# Autodesk Inventor assembly: 000 Ensamblaje hw_DAA - PCB Peripherals
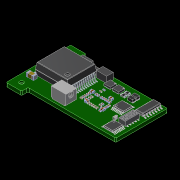
[picture p0: Inventor's stored thumbnail of the model, 180x180]
Saved by Autodesk Inventor 2018 (Build 220112000, 112)
## iProperties
Created: 2024-03-13
Part Number: 000 Ensamblaje hw_DAA - PCB Peripherals
Document SubType Name: Assembly
Designer: cda1
Author: cda1
## Documents named in this file (38)
- C:\Users\cda1\Git\DAA\items\hw_DAA\variants\BASIC\3d\000 Ensamblaje hw_DAA - PCB Peripherals.iam
- C:\Users\cda1\Git\DAA\items\hw_DAA\3d\hw_DAA - PCB Peripherals.ipt
- C:\Users\cda1\Git\DAA\items\_accessories\Componentes PCB\Drivers\3d_Texas Instruments\3d\SN65C3221IPWRQ1\SN65C3221IPWRQ1.iam
- C:\Users\cda1\Git\DAA\items\_accessories\Componentes PCB\Drivers\3d_Texas Instruments\3d\SN65HVD33MDREP\SN65HVD33MDREP.iam
- C:\Users\cda1\Git\DAA\items\_accessories\Componentes PCB\CAN\3d\3d_Texas_Instruments\TCAN1462VDRBRQ1\TCAN1462VDRBRQ1.iam
- C:\Users\cda1\Git\DAA\items\_accessories\Componentes PCB\Optoacoplador\3d_Toshiba\3d\TLP3431\TLP3431_TP,F.iam
- C:\Users\cda1\Git\DAA\items\_accessories\Componentes PCB\Optoacoplador\3d_Toshiba\3d\TLP3475(TP,F\TLP3475(TP,F.ipt
- C:\Users\cda1\Git\DAA\items\_accessories\Componentes PCB\Voltage-Level\3d\3d_Texas_Instruments\TXB0106IPWRQ1\TXB0106IPWRQ1.iam
- C:\Users\cda1\Git\DAA\items\_accessories\Componentes PCB\Filtro\3d_Coilcraft\1812CAN-113NRC\1812CAN-113NRC.iam
- C:\Users\cda1\Git\DAA\items\_accessories\Componentes PCB\Oscilador\3d_ECS_International\ECS-2520MVQ-250-CN-TR\ECS-2520MVQ-250-CN-TR.ipt
- C:\Users\cda1\Git\DAA\items\_accessories\Componentes PCB\Transceptor\3d_Texas Instrument\3d\DP83867ERGZT\DP83867ERGZT.iam
- C:\Users\cda1\Git\DAA\items\_accessories\Componentes PCB\Elementos mecanicos soldables\3d_Wurth Electronics\3d\SMD\WP-SMRA Redcube (M2) 746630200.ipt
- C:\Users\cda1\Git\DAA\items\_accessories\Componentes PCB\Resistencias\3d_Panasonic\3d\ERJ-P06F1200V\ERJ-P06F1200V.iam
- C:\Users\cda1\Git\DAA\items\_accessories\Componentes PCB\Capacitadores\3d_TDK\3d\CGA2B3X8R1H103K050BB.ipt
- C:\Users\cda1\Git\DAA\items\_accessories\Componentes PCB\Capacitadores\3d_Murata Electronics\3d\GRT155R61E105KE01D.ipt
- C:\Users\cda1\Git\DAA\items\_accessories\Componentes PCB\Capacitadores\3d_TDK\3d\CGA2B3X7R1H104K050BD.ipt
- C:\Users\cda1\Git\DAA\items\_accessories\Componentes PCB\Capacitadores\3d_Murata Electronics\3d\GRT188C81A106ME13D.ipt
- C:\Users\cda1\Git\DAA\items\_accessories\Componentes PCB\Capacitadores\3d_Murata Electronics\3d\NFM18HC106D0G3L\NFM18HC106D0G3L.ipt
- C:\Users\cda1\Git\DAA\items\_accessories\Componentes PCB\Resistencias\3d_Panasonic\3d\ERJ-2RKF1001X.ipt
- C:\Users\cda1\Git\DAA\items\_accessories\Componentes PCB\Diodos\3d_Diodes Incorporated\3d\DMG1012TQ-7\DMG1012TQ-7.iam
- C:\Users\cda1\Git\DAA\items\_accessories\Componentes PCB\Diodos\3d_Semtech\3d\RCLAMP3324PQTCT\RCLAMP3324PQTCT.ipt
- C:\Users\cda1\Git\DAA\items\_accessories\Componentes PCB\Diodos\3d_ST Microelectronics\HSP051-4M10\HSP051-4M10.ipt
- C:\Users\cda1\Git\DAA\items\_accessories\Componentes PCB\Resistencias\3d_Panasonic\3d\ERJ-2GE0R00X.ipt
- C:\Users\cda1\Git\DAA\items\_accessories\Componentes PCB\Resistencias\3d_Panasonic\3d\ERJ-2RKF1002X.ipt
- C:\Users\cda1\Git\DAA\items\_accessories\Componentes PCB\Resistencias\3d_Vishay\3d\CRCW0402499RFKEDHP\CRCW0402499RFKEDHP.iam
- C:\Users\cda1\Git\DAA\items\_accessories\Componentes PCB\Resistencias\3d_Genérico\RESC-0402.ipt
- C:\Users\cda1\Git\DAA\items\_accessories\Componentes PCB\Resistencias\3d_Vishay\3d\CRCW060310R0FKEAHP\CRCW060310R0FKEAHP.ipt
- C:\Users\cda1\Git\DAA\items\_accessories\Componentes PCB\Resistencias\3d_Panasonic\3d\ERJ-U02F2491X\ERJ-U02F2491X.iam
- C:\Users\cda1\Git\DAA\items\_accessories\Componentes PCB\Resistencias\3d_Vishay\3d\CRCW04025K76FKED\CRCW04025K76FKED.ipt
- C:\Users\cda1\Git\DAA\items\_accessories\Componentes PCB\Resistencias\3d_Vishay\3d\CRCW04022K20FKED\CRCW04022K20FKED.ipt
- C:\Users\cda1\Git\DAA\items\_accessories\Componentes PCB\Resistencias\3d_Panasonic\3d\ERJ-2RKF1501X.ipt
- C:\Users\cda1\Git\DAA\items\_accessories\Componentes PCB\Resistencias\3d_Panasonic\3d\ERJ-2RKF1102X\ERJ-2RKF1102X.iam
- C:\Users\cda1\Git\DAA\items\_accessories\Componentes PCB\Resistencias\3d_Panasonic\3d\ERJ-P06F60R4V.ipt
- C:\Users\cda1\Git\DAA\items\_accessories\Componentes PCB\Condensadores\3d-Murata\3d\GCM155R72A472MA37D\GCM155R72A472MA37D.ipt
- C:\Users\cda1\Git\DAA\items\_accessories\Componentes PCB\Resistencias\3d_Panasonic\3d\ERJ-2RKF75R0X\ERJ-2RKF75R0X.iam
- C:\Users\cda1\Git\DAA\items\_accessories\Componentes PCB\Capacitadores\3d_Kemet\3d\C1206C102KGRACAUTO\C1206C102KGRACAUTO.ipt
- C:\Users\cda1\Git\DAA\items\_accessories\Componentes PCB\Conectores\3d_Samtec\3d\CLP-105-02-F-D-BE\CLP-105-02-F-D-BE.iam
- C:\Users\cda1\Git\DAA\items\_accessories\Componentes PCB\Transformadores de señal\3d_Pulse_Electronics\HX5008NL\HX5008NL.iam
## Components (148 placed, 37 different names)
1. hw_DAA - PCB Peripherals:1 — Coincidencia:7, Coincidencia:8, Coincidencia:9, Coincidencia:10, Coincidencia:11, Coincidencia:12, Coincidencia:17, Coincidencia:18, Coincidencia:19, Coincidencia:20, Coincidencia:21, Coincidencia:22, Coincidencia:23, Coincidencia:24, Coincidencia:44, Ángulo:1, Ángulo:2, Ángulo:3, Ángulo:4, Ángulo:5, Coincidencia:45, Coincidencia:46, Coincidencia:47, Coincidencia:48, Coincidencia:49, Coincidencia:50, Coincidencia:51, Coincidencia:52, Coincidencia:53, Coincidencia:54, Coincidencia:55, Coincidencia:57, Coincidencia:58, Coincidencia:64, Coincidencia:65, Coincidencia:66, Coincidencia:67, Coincidencia:68, Coincidencia:71, Coincidencia:72, Ángulo:6, Coincidencia:73, Coincidencia:74, Coincidencia:75, Coincidencia:76, Coincidencia:77, Coincidencia:78, Coincidencia:79, Coincidencia:80, Coincidencia:81, Coincidencia:82, Coincidencia:83, Coincidencia:84, Coincidencia:85, Coincidencia:86, Coincidencia:87, Coincidencia:88, Coincidencia:89, Ángulo:7, Coincidencia:90, Coincidencia:91, Coincidencia:92, Coincidencia:93, Ángulo:8, Ángulo:9, Ángulo:10, Ángulo:11, Coincidencia:94, Coincidencia:95, Ángulo:12, Ángulo:13, Coincidencia:96, Coincidencia:97, Coincidencia:98, Coincidencia:99, Coincidencia:100, Coincidencia:101, Coincidencia:102, Coincidencia:103, Coincidencia:104, Coincidencia:105, Coincidencia:106, Ángulo:14, Coincidencia:107, Coincidencia:108, Coincidencia:109, Coincidencia:110, Ángulo:15, Ángulo:16, Coincidencia:111, Coincidencia:112, Coincidencia:113, Coincidencia:114, Coincidencia:115, Ángulo:17, Ángulo:18, Coincidencia:116, Coincidencia:117, Ángulo:19, Ángulo:20, Coincidencia:118, Coincidencia:119, Coincidencia:120, Coincidencia:121, Ángulo:21, Ángulo:22, Ángulo:23, Ángulo:24, Coincidencia:122, Ángulo:25, Coincidencia:123, Coincidencia:124, Coincidencia:125, Coincidencia:126, Coincidencia:127, Coincidencia:128, Coincidencia:129, Coincidencia:130, Coincidencia:131, Coincidencia:132, Coincidencia:133, Coincidencia:134, Ángulo:26, Ángulo:27, Coincidencia:135, Ángulo:28, Coincidencia:136, Ángulo:29, Coincidencia:137, Coincidencia:138, Coincidencia:139, Coincidencia:140, Ángulo:30, Ángulo:31, Coincidencia:141, Coincidencia:142, Ángulo:32, Ángulo:33, Coincidencia:143, Ángulo:34, Coincidencia:144, Ángulo:35, Coincidencia:145, Coincidencia:146, Coincidencia:147, Coincidencia:148, Coincidencia:149, Ángulo:36, Coincidencia:150, Ángulo:37, Coincidencia:151, Coincidencia:152, Coincidencia:153, Coincidencia:154, Coincidencia:155, Coincidencia:156, Coincidencia:157, Ángulo:38, Ángulo:39, Coincidencia:158, Ángulo:40, Coincidencia:159, Ángulo:41, Coincidencia:160, Ángulo:42, Coincidencia:161, Coincidencia:162, Coincidencia:163, Coincidencia:164, Coincidencia:165, Ángulo:43, Coincidencia:166, Coincidencia:167, Coincidencia:168, Coincidencia:169, Ángulo:44, Coincidencia:170, Coincidencia:171, Coincidencia:172, Coincidencia:173, Coincidencia:174, Coincidencia:175, Coincidencia:176, Coincidencia:178, Ángulo:45, Nivelación:1, Coincidencia:179, Ángulo:46, Coincidencia:180, Ángulo:47, Ángulo:48, Coincidencia:181, Ángulo:49, Ángulo:50, Ángulo:51, Coincidencia:182, Coincidencia:183, Coincidencia:184, Coincidencia:185, Coincidencia:186, Coincidencia:187, Ángulo:52, Ángulo:53
2. SN65C3221IPWRQ1:1 [sub-assembly] — Coincidencia:7, Coincidencia:8
3. SN65HVD33MDREP:1 [sub-assembly] — Coincidencia:9, Coincidencia:10
4. TCAN1462VDRBRQ1:1 [sub-assembly] — Coincidencia:11, Ángulo:2
5. TCAN1462VDRBRQ1:2 [sub-assembly] — Coincidencia:12, Ángulo:3
6. TLP3475(TP,F:1 — Coincidencia:17, Ángulo:5
7. TLP3475(TP,F:2 — Coincidencia:18, Ángulo:4
8. TXB0106IPWRQ1:1 [sub-assembly] — Coincidencia:19, Coincidencia:20
9. 1812CAN-113NRC:1 [sub-assembly] — Coincidencia:21
10. 1812CAN-113NRC:2 [sub-assembly] — Coincidencia:22
11. ECS-2520MVQ-250-CN-TR:1 — Coincidencia:23
12. DP83867ERGZT:1 [sub-assembly] — Coincidencia:24
13. WP-SMRA Redcube (M2) 746630200:1 — Coincidencia:44, Ángulo:1, Nivelación:1
14. TLP3431_TP,F:5 [sub-assembly] — Coincidencia:45
15. TLP3431_TP,F:6 [sub-assembly] — Coincidencia:46
16. TLP3431_TP,F:7 [sub-assembly] — Coincidencia:47
17. TLP3431_TP,F:8 [sub-assembly] — Coincidencia:48
18. ERJ-P06F1200V:1 [sub-assembly] — Coincidencia:49
19. ERJ-P06F1200V:2 [sub-assembly] — Coincidencia:50
20. CGA2B3X8R1H103K050BB:1 — Coincidencia:51
21. GRT155R61E105KE01D:1 — Coincidencia:52
22. CGA2B3X7R1H104K050BD:1 — Coincidencia:53
23. GRT155R61E105KE01D:2 — Coincidencia:54
24. CGA2B3X7R1H104K050BD:2 — Coincidencia:55
25. CGA2B3X8R1H103K050BB:2 — Ángulo:48
26. GRT188C81A106ME13D:1 — Coincidencia:57
27. GRT188C81A106ME13D:2 — Coincidencia:58, Ángulo:47
28. CGA2B3X7R1H104K050BD:3 — Coincidencia:185
29. CGA2B3X7R1H104K050BD:4 — Coincidencia:184
30. CGA2B3X7R1H104K050BD:5 — Coincidencia:183
31. CGA2B3X7R1H104K050BD:6 — Coincidencia:182
32. CGA2B3X7R1H104K050BD:8 — Coincidencia:64
33. CGA2B3X7R1H104K050BD:9 — Coincidencia:65
34. CGA2B3X7R1H104K050BD:10 — Coincidencia:66
35. CGA2B3X7R1H104K050BD:11 — Coincidencia:67
36. CGA2B3X7R1H104K050BD:12 — Coincidencia:68
37. NFM18HC106D0G3L:1 — Coincidencia:186
38. NFM18HC106D0G3L:2 — Coincidencia:187
39. CGA2B3X7R1H104K050BD:13 — Coincidencia:72
40. CGA2B3X7R1H104K050BD:14 — Coincidencia:71
41. GRT155R61E105KE01D:3 — Ángulo:6, Coincidencia:73
42. GRT155R61E105KE01D:4 — Coincidencia:74
43. GRT155R61E105KE01D:5 — Coincidencia:75
44. GRT155R61E105KE01D:6 — Coincidencia:76
45. GRT155R61E105KE01D:7 — Coincidencia:77
46. GRT155R61E105KE01D:8 — Coincidencia:78
47. GRT155R61E105KE01D:9 — Coincidencia:79
48. GRT155R61E105KE01D:10 — Coincidencia:80
49. CGA2B3X7R1H104K050BD:15 — Coincidencia:81
50. CGA2B3X7R1H104K050BD:16 — Coincidencia:82
51. GRT155R61E105KE01D:11 — Coincidencia:83
52. CGA2B3X8R1H103K050BB:3 — Coincidencia:84
53. GRT188C81A106ME13D:3 — Coincidencia:85
54. GRT188C81A106ME13D:4 — Coincidencia:86
55. CGA2B3X7R1H104K050BD:17 — Coincidencia:87
56. ERJ-2RKF1001X:1 — Coincidencia:88
57. NFM18HC106D0G3L:3 — Coincidencia:89, Ángulo:7
58. DMG1012TQ-7:5 [sub-assembly] — Coincidencia:93, Ángulo:9
59. DMG1012TQ-7:6 [sub-assembly] — Coincidencia:92, Ángulo:8
60. DMG1012TQ-7:7 [sub-assembly] — Coincidencia:91, Ángulo:11
61. DMG1012TQ-7:8 [sub-assembly] — Coincidencia:90, Ángulo:10
62. RCLAMP3324PQTCT:1 — Coincidencia:94, Ángulo:13
63. RCLAMP3324PQTCT:2 — Coincidencia:95, Ángulo:12
64. HSP051-4M10:1 — Coincidencia:97
65. HSP051-4M10:2 — Coincidencia:96
66. ERJ-2GE0R00X:1 — Coincidencia:98
67. ERJ-2GE0R00X:2 — Coincidencia:99
68. ERJ-2GE0R00X:3 — Coincidencia:100
69. ERJ-2GE0R00X:4 — Coincidencia:101
70. ERJ-2GE0R00X:5 — Coincidencia:102
71. ERJ-2GE0R00X:6 — Coincidencia:103
72. CGA2B3X7R1H104K050BD:18 — Coincidencia:104
73. ERJ-2RKF1002X:1 — Coincidencia:105
74. CGA2B3X7R1H104K050BD:19 — Coincidencia:106, Ángulo:14
75. CGA2B3X7R1H104K050BD:20 — Coincidencia:107
76. ERJ-2RKF1002X:2 — Coincidencia:108
77. ERJ-2RKF1002X:3 — Coincidencia:109, Ángulo:15
78. ERJ-2RKF1002X:4 — Coincidencia:110, Ángulo:16
79. CGA2B3X7R1H104K050BD:21 — Coincidencia:111
80. ERJ-2RKF1002X:5 — Coincidencia:112
81. ERJ-2RKF1002X:6 — Coincidencia:113
82. CRCW0402499RFKEDHP:1 [sub-assembly] — Coincidencia:114, Ángulo:18
83. CRCW0402499RFKEDHP:2 [sub-assembly] — Coincidencia:115, Ángulo:17
84. RESC-0402:1 — Coincidencia:116, Ángulo:19
85. RESC-0402:2 — Coincidencia:117, Ángulo:20
86. CRCW060310R0FKEAHP:1 — Coincidencia:118, Ángulo:21
87. CRCW060310R0FKEAHP:2 — Coincidencia:119, Ángulo:23
88. CRCW060310R0FKEAHP:3 — Coincidencia:120, Ángulo:22
89. CRCW060310R0FKEAHP:4 — Coincidencia:121, Ángulo:24
90. NFM18HC106D0G3L:4 — Coincidencia:122, Ángulo:25
91. ERJ-2RKF1002X:7 — Coincidencia:123
92. ERJ-2RKF1002X:8 — Coincidencia:124
93. ERJ-2RKF1002X:9 — Coincidencia:125
94. CGA2B3X7R1H104K050BD:22 — Coincidencia:126
95. CGA2B3X7R1H104K050BD:23 — Coincidencia:127
96. CGA2B3X7R1H104K050BD:24 — Coincidencia:128
97. CGA2B3X7R1H104K050BD:25 — Coincidencia:129
98. ERJ-2RKF1002X:10 — Coincidencia:130
99. ERJ-U02F2491X:1 [sub-assembly] — Coincidencia:131
100. RESC-0402:3 — Coincidencia:132
101. ERJ-U02F2491X:2 [sub-assembly] — Coincidencia:133, Ángulo:26
102. RESC-0402:4 — Coincidencia:134, Ángulo:27
103. CRCW04025K76FKED:1 — Coincidencia:135, Ángulo:28
104. ERJ-U02F2491X:3 [sub-assembly] — Coincidencia:136, Ángulo:29
105. RESC-0402:5 — Coincidencia:138, Ángulo:50
106. RESC-0402:6 — Coincidencia:137, Ángulo:49
107. RESC-0402:7 — Coincidencia:139, Ángulo:30
108. RESC-0402:8 — Coincidencia:140, Ángulo:31
109. CRCW04022K20FKED:1 — Coincidencia:141, Ángulo:32
110. CRCW04022K20FKED:2 — Coincidencia:142, Ángulo:33
111. ERJ-2RKF1002X:11 — Coincidencia:143, Ángulo:34
112. ERJ-U02F2491X:4 [sub-assembly] — Coincidencia:144, Ángulo:35
113. RESC-0402:9 — Coincidencia:145
114. RESC-0402:10 — Coincidencia:147
115. RESC-0402:11 — Coincidencia:148
116. RESC-0402:12 — Coincidencia:146
117. CGA2B3X8R1H103K050BB:4 — Coincidencia:149, Ángulo:36
118. ERJ-2RKF1002X:12 — Coincidencia:150, Ángulo:37
119. ERJ-2RKF1002X:13 — Coincidencia:151
120. ERJ-2RKF1002X:14 — Coincidencia:152
121. ERJ-2RKF1002X:15 — Coincidencia:153
122. CGA2B3X7R1H104K050BD:26 — Coincidencia:154
123. CGA2B3X7R1H104K050BD:27 — Coincidencia:155
124. CGA2B3X7R1H104K050BD:28 — Coincidencia:156, Ángulo:38
125. CGA2B3X7R1H104K050BD:29 — Coincidencia:157, Ángulo:39
126. ERJ-2RKF1501X:1 — Coincidencia:158, Ángulo:40
127. ERJ-2RKF1102X:1 [sub-assembly] — Coincidencia:159, Ángulo:41
128. RESC-0402:13 — Coincidencia:160, Ángulo:42
129. ERJ-P06F60R4V:1 — Coincidencia:161
130. ERJ-P06F60R4V:2 — Coincidencia:162
131. ERJ-P06F60R4V:3 — Coincidencia:164
132. ERJ-P06F60R4V:4 — Coincidencia:163
133. ERJ-2RKF1002X:16 — Coincidencia:165, Ángulo:43
134. GCM155R72A472MA37D:1 — Coincidencia:166, Ángulo:51
135. CRCW0402499RFKEDHP:3 [sub-assembly] — Coincidencia:168
136. CRCW0402499RFKEDHP:4 [sub-assembly] — Coincidencia:167
137. ERJ-2RKF1002X:17 — Coincidencia:169, Ángulo:44
138. GCM155R72A472MA37D:2 — Coincidencia:170
139. CRCW0402499RFKEDHP:5 [sub-assembly] — Coincidencia:171, Ángulo:53
140. CRCW0402499RFKEDHP:6 [sub-assembly] — Coincidencia:172, Ángulo:52
141. ERJ-2RKF75R0X:1 [sub-assembly] — Coincidencia:173
142. ERJ-2RKF75R0X:2 [sub-assembly] — Coincidencia:174
143. ERJ-2RKF75R0X:3 [sub-assembly] — Coincidencia:175
144. ERJ-2RKF75R0X:4 [sub-assembly] — Coincidencia:176
145. C1206C102KGRACAUTO:1 — Coincidencia:180
146. CLP-105-02-F-D-BE:1 [sub-assembly] — Coincidencia:178, Ángulo:45
147. HX5008NL:1 [sub-assembly] — Coincidencia:179, Ángulo:46
148. GRT155R61E105KE01D:12 — Coincidencia:181
## Relationships (203: Mate 149, Angle 53, Flush 1)
- Coincidencia:7 [Mate]: hw_DAA - PCB Peripherals:1 ↔ SN65C3221IPWRQ1:1
- Coincidencia:8 [Mate]: hw_DAA - PCB Peripherals:1 ↔ SN65C3221IPWRQ1:1
- Coincidencia:9 [Mate]: hw_DAA - PCB Peripherals:1 ↔ SN65HVD33MDREP:1
- Coincidencia:10 [Mate]: hw_DAA - PCB Peripherals:1 ↔ SN65HVD33MDREP:1
- Coincidencia:11 [Mate]: hw_DAA - PCB Peripherals:1 ↔ TCAN1462VDRBRQ1:1
- Coincidencia:12 [Mate]: hw_DAA - PCB Peripherals:1 ↔ TCAN1462VDRBRQ1:2
- Coincidencia:17 [Mate]: hw_DAA - PCB Peripherals:1 ↔ TLP3475(TP,F:1
- Coincidencia:18 [Mate]: hw_DAA - PCB Peripherals:1 ↔ TLP3475(TP,F:2
- Coincidencia:19 [Mate]: hw_DAA - PCB Peripherals:1 ↔ TXB0106IPWRQ1:1
- Coincidencia:20 [Mate]: hw_DAA - PCB Peripherals:1 ↔ TXB0106IPWRQ1:1
- Coincidencia:21 [Mate]: hw_DAA - PCB Peripherals:1 ↔ 1812CAN-113NRC:1
- Coincidencia:22 [Mate]: hw_DAA - PCB Peripherals:1 ↔ 1812CAN-113NRC:2
- Coincidencia:23 [Mate]: hw_DAA - PCB Peripherals:1 ↔ ECS-2520MVQ-250-CN-TR:1
- Coincidencia:24 [Mate]: hw_DAA - PCB Peripherals:1 ↔ DP83867ERGZT:1
- Coincidencia:44 [Mate]: hw_DAA - PCB Peripherals:1 ↔ WP-SMRA Redcube (M2) 746630200:1
- Ángulo:1 [Angle] (0 deg): hw_DAA - PCB Peripherals:1 ↔ WP-SMRA Redcube (M2) 746630200:1
- Ángulo:2 [Angle] (0 deg): hw_DAA - PCB Peripherals:1 ↔ TCAN1462VDRBRQ1:1
- Ángulo:3 [Angle] (0 deg): hw_DAA - PCB Peripherals:1 ↔ TCAN1462VDRBRQ1:2
- Ángulo:4 [Angle] (0 deg): hw_DAA - PCB Peripherals:1 ↔ TLP3475(TP,F:2
- Ángulo:5 [Angle] (0 deg): hw_DAA - PCB Peripherals:1 ↔ TLP3475(TP,F:1
- Coincidencia:45 [Mate]: hw_DAA - PCB Peripherals:1 ↔ TLP3431_TP,F:5
- Coincidencia:46 [Mate]: hw_DAA - PCB Peripherals:1 ↔ TLP3431_TP,F:6
- Coincidencia:47 [Mate]: hw_DAA - PCB Peripherals:1 ↔ TLP3431_TP,F:7
- Coincidencia:48 [Mate]: hw_DAA - PCB Peripherals:1 ↔ TLP3431_TP,F:8
- Coincidencia:49 [Mate]: hw_DAA - PCB Peripherals:1 ↔ ERJ-P06F1200V:1
- Coincidencia:50 [Mate]: hw_DAA - PCB Peripherals:1 ↔ ERJ-P06F1200V:2
- Coincidencia:51 [Mate]: hw_DAA - PCB Peripherals:1 ↔ CGA2B3X8R1H103K050BB:1
- Coincidencia:52 [Mate]: hw_DAA - PCB Peripherals:1 ↔ GRT155R61E105KE01D:1
- Coincidencia:53 [Mate]: hw_DAA - PCB Peripherals:1 ↔ CGA2B3X7R1H104K050BD:1
- Coincidencia:54 [Mate]: hw_DAA - PCB Peripherals:1 ↔ GRT155R61E105KE01D:2
- Coincidencia:55 [Mate]: hw_DAA - PCB Peripherals:1 ↔ CGA2B3X7R1H104K050BD:2
- Coincidencia:57 [Mate]: hw_DAA - PCB Peripherals:1 ↔ GRT188C81A106ME13D:1
- Coincidencia:58 [Mate]: hw_DAA - PCB Peripherals:1 ↔ GRT188C81A106ME13D:2
- Coincidencia:64 [Mate]: hw_DAA - PCB Peripherals:1 ↔ CGA2B3X7R1H104K050BD:8
- Coincidencia:65 [Mate]: hw_DAA - PCB Peripherals:1 ↔ CGA2B3X7R1H104K050BD:9
- Coincidencia:66 [Mate]: hw_DAA - PCB Peripherals:1 ↔ CGA2B3X7R1H104K050BD:10
- Coincidencia:67 [Mate]: hw_DAA - PCB Peripherals:1 ↔ CGA2B3X7R1H104K050BD:11
- Coincidencia:68 [Mate]: hw_DAA - PCB Peripherals:1 ↔ CGA2B3X7R1H104K050BD:12
- Coincidencia:71 [Mate]: hw_DAA - PCB Peripherals:1 ↔ CGA2B3X7R1H104K050BD:14
- Coincidencia:72 [Mate]: hw_DAA - PCB Peripherals:1 ↔ CGA2B3X7R1H104K050BD:13
- Ángulo:6 [Angle] (0 deg): hw_DAA - PCB Peripherals:1 ↔ GRT155R61E105KE01D:3
- Coincidencia:73 [Mate]: hw_DAA - PCB Peripherals:1 ↔ GRT155R61E105KE01D:3
- Coincidencia:74 [Mate]: hw_DAA - PCB Peripherals:1 ↔ GRT155R61E105KE01D:4
- Coincidencia:75 [Mate]: hw_DAA - PCB Peripherals:1 ↔ GRT155R61E105KE01D:5
- Coincidencia:76 [Mate]: hw_DAA - PCB Peripherals:1 ↔ GRT155R61E105KE01D:6
- Coincidencia:77 [Mate]: hw_DAA - PCB Peripherals:1 ↔ GRT155R61E105KE01D:7
- Coincidencia:78 [Mate]: hw_DAA - PCB Peripherals:1 ↔ GRT155R61E105KE01D:8
- Coincidencia:79 [Mate]: hw_DAA - PCB Peripherals:1 ↔ GRT155R61E105KE01D:9
- Coincidencia:80 [Mate]: hw_DAA - PCB Peripherals:1 ↔ GRT155R61E105KE01D:10
- Coincidencia:81 [Mate]: hw_DAA - PCB Peripherals:1 ↔ CGA2B3X7R1H104K050BD:15
- Coincidencia:82 [Mate]: hw_DAA - PCB Peripherals:1 ↔ CGA2B3X7R1H104K050BD:16
- Coincidencia:83 [Mate]: hw_DAA - PCB Peripherals:1 ↔ GRT155R61E105KE01D:11
- Coincidencia:84 [Mate]: hw_DAA - PCB Peripherals:1 ↔ CGA2B3X8R1H103K050BB:3
- Coincidencia:85 [Mate]: hw_DAA - PCB Peripherals:1 ↔ GRT188C81A106ME13D:3
- Coincidencia:86 [Mate]: hw_DAA - PCB Peripherals:1 ↔ GRT188C81A106ME13D:4
- Coincidencia:87 [Mate]: hw_DAA - PCB Peripherals:1 ↔ CGA2B3X7R1H104K050BD:17
- Coincidencia:88 [Mate]: hw_DAA - PCB Peripherals:1 ↔ ERJ-2RKF1001X:1
- Coincidencia:89 [Mate]: hw_DAA - PCB Peripherals:1 ↔ NFM18HC106D0G3L:3
- Ángulo:7 [Angle] (0 deg): hw_DAA - PCB Peripherals:1 ↔ NFM18HC106D0G3L:3
- Coincidencia:90 [Mate]: hw_DAA - PCB Peripherals:1 ↔ DMG1012TQ-7:8
- Coincidencia:91 [Mate]: hw_DAA - PCB Peripherals:1 ↔ DMG1012TQ-7:7
- Coincidencia:92 [Mate]: hw_DAA - PCB Peripherals:1 ↔ DMG1012TQ-7:6
- Coincidencia:93 [Mate]: hw_DAA - PCB Peripherals:1 ↔ DMG1012TQ-7:5
- Ángulo:8 [Angle] (0 deg): hw_DAA - PCB Peripherals:1 ↔ DMG1012TQ-7:6
- Ángulo:9 [Angle] (0 deg): hw_DAA - PCB Peripherals:1 ↔ DMG1012TQ-7:5
- Ángulo:10 [Angle] (0 deg): hw_DAA - PCB Peripherals:1 ↔ DMG1012TQ-7:8
- Ángulo:11 [Angle] (0 deg): hw_DAA - PCB Peripherals:1 ↔ DMG1012TQ-7:7
- Coincidencia:94 [Mate]: hw_DAA - PCB Peripherals:1 ↔ RCLAMP3324PQTCT:1
- Coincidencia:95 [Mate]: hw_DAA - PCB Peripherals:1 ↔ RCLAMP3324PQTCT:2
- Ángulo:12 [Angle] (0 deg): hw_DAA - PCB Peripherals:1 ↔ RCLAMP3324PQTCT:2
- Ángulo:13 [Angle] (0 deg): hw_DAA - PCB Peripherals:1 ↔ RCLAMP3324PQTCT:1
- Coincidencia:96 [Mate]: hw_DAA - PCB Peripherals:1 ↔ HSP051-4M10:2
- Coincidencia:97 [Mate]: hw_DAA - PCB Peripherals:1 ↔ HSP051-4M10:1
- Coincidencia:98 [Mate]: hw_DAA - PCB Peripherals:1 ↔ ERJ-2GE0R00X:1
- Coincidencia:99 [Mate]: hw_DAA - PCB Peripherals:1 ↔ ERJ-2GE0R00X:2
- Coincidencia:100 [Mate]: hw_DAA - PCB Peripherals:1 ↔ ERJ-2GE0R00X:3
- Coincidencia:101 [Mate]: hw_DAA - PCB Peripherals:1 ↔ ERJ-2GE0R00X:4
- Coincidencia:102 [Mate]: hw_DAA - PCB Peripherals:1 ↔ ERJ-2GE0R00X:5
- Coincidencia:103 [Mate]: hw_DAA - PCB Peripherals:1 ↔ ERJ-2GE0R00X:6
- Coincidencia:104 [Mate]: hw_DAA - PCB Peripherals:1 ↔ CGA2B3X7R1H104K050BD:18
- Coincidencia:105 [Mate]: hw_DAA - PCB Peripherals:1 ↔ ERJ-2RKF1002X:1
- Coincidencia:106 [Mate]: hw_DAA - PCB Peripherals:1 ↔ CGA2B3X7R1H104K050BD:19
- Ángulo:14 [Angle] (0 deg): hw_DAA - PCB Peripherals:1 ↔ CGA2B3X7R1H104K050BD:19
- Coincidencia:107 [Mate]: hw_DAA - PCB Peripherals:1 ↔ CGA2B3X7R1H104K050BD:20
- Coincidencia:108 [Mate]: hw_DAA - PCB Peripherals:1 ↔ ERJ-2RKF1002X:2
- Coincidencia:109 [Mate]: hw_DAA - PCB Peripherals:1 ↔ ERJ-2RKF1002X:3
- Coincidencia:110 [Mate]: hw_DAA - PCB Peripherals:1 ↔ ERJ-2RKF1002X:4
- Ángulo:15 [Angle] (0 deg): hw_DAA - PCB Peripherals:1 ↔ ERJ-2RKF1002X:3
- Ángulo:16 [Angle] (0 deg): hw_DAA - PCB Peripherals:1 ↔ ERJ-2RKF1002X:4
- Coincidencia:111 [Mate]: hw_DAA - PCB Peripherals:1 ↔ CGA2B3X7R1H104K050BD:21
- Coincidencia:112 [Mate]: hw_DAA - PCB Peripherals:1 ↔ ERJ-2RKF1002X:5
- Coincidencia:113 [Mate]: hw_DAA - PCB Peripherals:1 ↔ ERJ-2RKF1002X:6
- Coincidencia:114 [Mate]: hw_DAA - PCB Peripherals:1 ↔ CRCW0402499RFKEDHP:1
- Coincidencia:115 [Mate]: hw_DAA - PCB Peripherals:1 ↔ CRCW0402499RFKEDHP:2
- Ángulo:17 [Angle] (0 deg): hw_DAA - PCB Peripherals:1 ↔ CRCW0402499RFKEDHP:2
- Ángulo:18 [Angle] (0 deg): hw_DAA - PCB Peripherals:1 ↔ CRCW0402499RFKEDHP:1
- Coincidencia:116 [Mate]: hw_DAA - PCB Peripherals:1 ↔ RESC-0402:1
- Coincidencia:117 [Mate]: hw_DAA - PCB Peripherals:1 ↔ RESC-0402:2
- Ángulo:19 [Angle] (0 deg): hw_DAA - PCB Peripherals:1 ↔ RESC-0402:1
- Ángulo:20 [Angle] (0 deg): hw_DAA - PCB Peripherals:1 ↔ RESC-0402:2
- Coincidencia:118 [Mate]: hw_DAA - PCB Peripherals:1 ↔ CRCW060310R0FKEAHP:1
- Coincidencia:119 [Mate]: hw_DAA - PCB Peripherals:1 ↔ CRCW060310R0FKEAHP:2
- Coincidencia:120 [Mate]: hw_DAA - PCB Peripherals:1 ↔ CRCW060310R0FKEAHP:3
- Coincidencia:121 [Mate]: hw_DAA - PCB Peripherals:1 ↔ CRCW060310R0FKEAHP:4
- Ángulo:21 [Angle] (0 deg): hw_DAA - PCB Peripherals:1 ↔ CRCW060310R0FKEAHP:1
- Ángulo:22 [Angle] (0 deg): hw_DAA - PCB Peripherals:1 ↔ CRCW060310R0FKEAHP:3
- Ángulo:23 [Angle] (0 deg): hw_DAA - PCB Peripherals:1 ↔ CRCW060310R0FKEAHP:2
- Ángulo:24 [Angle] (0 deg): hw_DAA - PCB Peripherals:1 ↔ CRCW060310R0FKEAHP:4
- Coincidencia:122 [Mate]: hw_DAA - PCB Peripherals:1 ↔ NFM18HC106D0G3L:4
- Ángulo:25 [Angle] (0 deg): hw_DAA - PCB Peripherals:1 ↔ NFM18HC106D0G3L:4
- Coincidencia:123 [Mate]: hw_DAA - PCB Peripherals:1 ↔ ERJ-2RKF1002X:7
- Coincidencia:124 [Mate]: hw_DAA - PCB Peripherals:1 ↔ ERJ-2RKF1002X:8
- Coincidencia:125 [Mate]: hw_DAA - PCB Peripherals:1 ↔ ERJ-2RKF1002X:9
- Coincidencia:126 [Mate]: hw_DAA - PCB Peripherals:1 ↔ CGA2B3X7R1H104K050BD:22
- Coincidencia:127 [Mate]: hw_DAA - PCB Peripherals:1 ↔ CGA2B3X7R1H104K050BD:23
- Coincidencia:128 [Mate]: hw_DAA - PCB Peripherals:1 ↔ CGA2B3X7R1H104K050BD:24
- Coincidencia:129 [Mate]: hw_DAA - PCB Peripherals:1 ↔ CGA2B3X7R1H104K050BD:25
- Coincidencia:130 [Mate]: hw_DAA - PCB Peripherals:1 ↔ ERJ-2RKF1002X:10
- Coincidencia:131 [Mate]: hw_DAA - PCB Peripherals:1 ↔ ERJ-U02F2491X:1
- Coincidencia:132 [Mate]: hw_DAA - PCB Peripherals:1 ↔ RESC-0402:3
- Coincidencia:133 [Mate]: hw_DAA - PCB Peripherals:1 ↔ ERJ-U02F2491X:2
- Coincidencia:134 [Mate]: hw_DAA - PCB Peripherals:1 ↔ RESC-0402:4
- Ángulo:26 [Angle] (0 deg): hw_DAA - PCB Peripherals:1 ↔ ERJ-U02F2491X:2
- Ángulo:27 [Angle] (0 deg): hw_DAA - PCB Peripherals:1 ↔ RESC-0402:4
- Coincidencia:135 [Mate]: hw_DAA - PCB Peripherals:1 ↔ CRCW04025K76FKED:1
- Ángulo:28 [Angle] (0 deg): hw_DAA - PCB Peripherals:1 ↔ CRCW04025K76FKED:1
- Coincidencia:136 [Mate]: hw_DAA - PCB Peripherals:1 ↔ ERJ-U02F2491X:3
- Ángulo:29 [Angle] (0 deg): hw_DAA - PCB Peripherals:1 ↔ ERJ-U02F2491X:3
- Coincidencia:137 [Mate]: hw_DAA - PCB Peripherals:1 ↔ RESC-0402:6
- Coincidencia:138 [Mate]: hw_DAA - PCB Peripherals:1 ↔ RESC-0402:5
- Coincidencia:139 [Mate]: hw_DAA - PCB Peripherals:1 ↔ RESC-0402:7
- Coincidencia:140 [Mate]: hw_DAA - PCB Peripherals:1 ↔ RESC-0402:8
- Ángulo:30 [Angle] (0 deg): hw_DAA - PCB Peripherals:1 ↔ RESC-0402:7
- Ángulo:31 [Angle] (0 deg): hw_DAA - PCB Peripherals:1 ↔ RESC-0402:8
- Coincidencia:141 [Mate]: hw_DAA - PCB Peripherals:1 ↔ CRCW04022K20FKED:1
- Coincidencia:142 [Mate]: hw_DAA - PCB Peripherals:1 ↔ CRCW04022K20FKED:2
- Ángulo:32 [Angle] (0 deg): hw_DAA - PCB Peripherals:1 ↔ CRCW04022K20FKED:1
- Ángulo:33 [Angle] (0 deg): hw_DAA - PCB Peripherals:1 ↔ CRCW04022K20FKED:2
- Coincidencia:143 [Mate]: hw_DAA - PCB Peripherals:1 ↔ ERJ-2RKF1002X:11
- Ángulo:34 [Angle] (0 deg): hw_DAA - PCB Peripherals:1 ↔ ERJ-2RKF1002X:11
- Coincidencia:144 [Mate]: hw_DAA - PCB Peripherals:1 ↔ ERJ-U02F2491X:4
- Ángulo:35 [Angle] (0 deg): hw_DAA - PCB Peripherals:1 ↔ ERJ-U02F2491X:4
- Coincidencia:145 [Mate]: hw_DAA - PCB Peripherals:1 ↔ RESC-0402:9
- Coincidencia:146 [Mate]: hw_DAA - PCB Peripherals:1 ↔ RESC-0402:12
- Coincidencia:147 [Mate]: hw_DAA - PCB Peripherals:1 ↔ RESC-0402:10
- Coincidencia:148 [Mate]: hw_DAA - PCB Peripherals:1 ↔ RESC-0402:11
- Coincidencia:149 [Mate]: hw_DAA - PCB Peripherals:1 ↔ CGA2B3X8R1H103K050BB:4
- Ángulo:36 [Angle] (0 deg): hw_DAA - PCB Peripherals:1 ↔ CGA2B3X8R1H103K050BB:4
- Coincidencia:150 [Mate]: hw_DAA - PCB Peripherals:1 ↔ ERJ-2RKF1002X:12
- Ángulo:37 [Angle] (0 deg): hw_DAA - PCB Peripherals:1 ↔ ERJ-2RKF1002X:12
- Coincidencia:151 [Mate]: hw_DAA - PCB Peripherals:1 ↔ ERJ-2RKF1002X:13
- Coincidencia:152 [Mate]: hw_DAA - PCB Peripherals:1 ↔ ERJ-2RKF1002X:14
- Coincidencia:153 [Mate]: hw_DAA - PCB Peripherals:1 ↔ ERJ-2RKF1002X:15
- Coincidencia:154 [Mate]: hw_DAA - PCB Peripherals:1 ↔ CGA2B3X7R1H104K050BD:26
- Coincidencia:155 [Mate]: hw_DAA - PCB Peripherals:1 ↔ CGA2B3X7R1H104K050BD:27
- Coincidencia:156 [Mate]: hw_DAA - PCB Peripherals:1 ↔ CGA2B3X7R1H104K050BD:28
- Coincidencia:157 [Mate]: hw_DAA - PCB Peripherals:1 ↔ CGA2B3X7R1H104K050BD:29
- Ángulo:38 [Angle] (0 deg): hw_DAA - PCB Peripherals:1 ↔ CGA2B3X7R1H104K050BD:28
- Ángulo:39 [Angle] (0 deg): hw_DAA - PCB Peripherals:1 ↔ CGA2B3X7R1H104K050BD:29
- Coincidencia:158 [Mate]: hw_DAA - PCB Peripherals:1 ↔ ERJ-2RKF1501X:1
- Ángulo:40 [Angle] (0 deg): hw_DAA - PCB Peripherals:1 ↔ ERJ-2RKF1501X:1
- Coincidencia:159 [Mate]: hw_DAA - PCB Peripherals:1 ↔ ERJ-2RKF1102X:1
- Ángulo:41 [Angle] (0 deg): hw_DAA - PCB Peripherals:1 ↔ ERJ-2RKF1102X:1
- Coincidencia:160 [Mate]: hw_DAA - PCB Peripherals:1 ↔ RESC-0402:13
- Ángulo:42 [Angle] (0 deg): hw_DAA - PCB Peripherals:1 ↔ RESC-0402:13
- Coincidencia:161 [Mate]: hw_DAA - PCB Peripherals:1 ↔ ERJ-P06F60R4V:1
- Coincidencia:162 [Mate]: hw_DAA - PCB Peripherals:1 ↔ ERJ-P06F60R4V:2
- Coincidencia:163 [Mate]: hw_DAA - PCB Peripherals:1 ↔ ERJ-P06F60R4V:4
- Coincidencia:164 [Mate]: hw_DAA - PCB Peripherals:1 ↔ ERJ-P06F60R4V:3
- Coincidencia:165 [Mate]: hw_DAA - PCB Peripherals:1 ↔ ERJ-2RKF1002X:16
- Ángulo:43 [Angle] (0 deg): hw_DAA - PCB Peripherals:1 ↔ ERJ-2RKF1002X:16
- Coincidencia:166 [Mate]: hw_DAA - PCB Peripherals:1 ↔ GCM155R72A472MA37D:1
- Coincidencia:167 [Mate]: hw_DAA - PCB Peripherals:1 ↔ CRCW0402499RFKEDHP:4
- Coincidencia:168 [Mate]: hw_DAA - PCB Peripherals:1 ↔ CRCW0402499RFKEDHP:3
- Coincidencia:169 [Mate]: hw_DAA - PCB Peripherals:1 ↔ ERJ-2RKF1002X:17
- Ángulo:44 [Angle] (0 deg): hw_DAA - PCB Peripherals:1 ↔ ERJ-2RKF1002X:17
- Coincidencia:170 [Mate]: hw_DAA - PCB Peripherals:1 ↔ GCM155R72A472MA37D:2
- Coincidencia:171 [Mate]: hw_DAA - PCB Peripherals:1 ↔ CRCW0402499RFKEDHP:5
- Coincidencia:172 [Mate]: hw_DAA - PCB Peripherals:1 ↔ CRCW0402499RFKEDHP:6
- Coincidencia:173 [Mate]: hw_DAA - PCB Peripherals:1 ↔ ERJ-2RKF75R0X:1
- Coincidencia:174 [Mate]: hw_DAA - PCB Peripherals:1 ↔ ERJ-2RKF75R0X:2
- Coincidencia:175 [Mate]: hw_DAA - PCB Peripherals:1 ↔ ERJ-2RKF75R0X:3
- Coincidencia:176 [Mate]: hw_DAA - PCB Peripherals:1 ↔ ERJ-2RKF75R0X:4
- Coincidencia:178 [Mate]: hw_DAA - PCB Peripherals:1 ↔ CLP-105-02-F-D-BE:1
- Ángulo:45 [Angle] (0 deg): hw_DAA - PCB Peripherals:1 ↔ CLP-105-02-F-D-BE:1
- Nivelación:1 [Flush] (24.692 mm): hw_DAA - PCB Peripherals:1 ↔ WP-SMRA Redcube (M2) 746630200:1
- Coincidencia:179 [Mate]: hw_DAA - PCB Peripherals:1 ↔ HX5008NL:1
- Ángulo:46 [Angle] (0 deg): hw_DAA - PCB Peripherals:1 ↔ HX5008NL:1
- Coincidencia:180 [Mate]: hw_DAA - PCB Peripherals:1 ↔ C1206C102KGRACAUTO:1
- Ángulo:47 [Angle] (0 deg): hw_DAA - PCB Peripherals:1 ↔ GRT188C81A106ME13D:2
- Ángulo:48 [Angle] (0 deg): hw_DAA - PCB Peripherals:1 ↔ CGA2B3X8R1H103K050BB:2
- Coincidencia:181 [Mate]: hw_DAA - PCB Peripherals:1 ↔ GRT155R61E105KE01D:12
- Ángulo:49 [Angle] (0 deg): hw_DAA - PCB Peripherals:1 ↔ RESC-0402:6
- Ángulo:50 [Angle] (0 deg): hw_DAA - PCB Peripherals:1 ↔ RESC-0402:5
- Ángulo:51 [Angle] (0 deg): hw_DAA - PCB Peripherals:1 ↔ GCM155R72A472MA37D:1
- Coincidencia:182 [Mate]: hw_DAA - PCB Peripherals:1 ↔ CGA2B3X7R1H104K050BD:6
- Coincidencia:183 [Mate]: hw_DAA - PCB Peripherals:1 ↔ CGA2B3X7R1H104K050BD:5
- Coincidencia:184 [Mate]: hw_DAA - PCB Peripherals:1 ↔ CGA2B3X7R1H104K050BD:4
- Coincidencia:185 [Mate]: hw_DAA - PCB Peripherals:1 ↔ CGA2B3X7R1H104K050BD:3
- Coincidencia:186 [Mate]: hw_DAA - PCB Peripherals:1 ↔ NFM18HC106D0G3L:1
- Coincidencia:187 [Mate]: hw_DAA - PCB Peripherals:1 ↔ NFM18HC106D0G3L:2
- Ángulo:52 [Angle] (0 deg): hw_DAA - PCB Peripherals:1 ↔ CRCW0402499RFKEDHP:6
- Ángulo:53 [Angle] (0 deg): hw_DAA - PCB Peripherals:1 ↔ CRCW0402499RFKEDHP:5
